# Autodesk Inventor assembly: мультипликатор
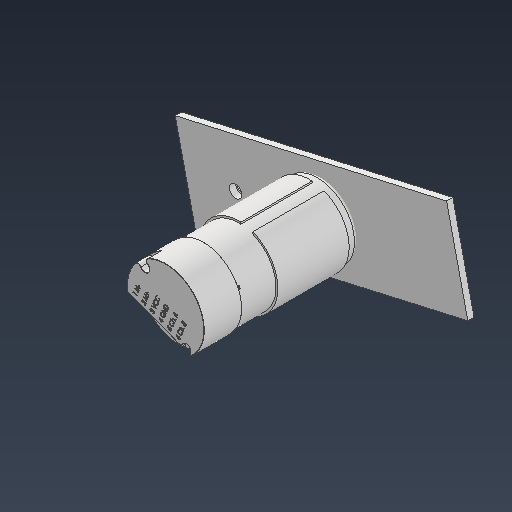
[picture p0: Inventor's stored thumbnail of the model, 512x512]
Saved by Autodesk Inventor 2025 (Build 290162000, 162)
## iProperties
Created: 2025-09-21
Part Number: мультипликатор
Document SubType Name: Assembly
Designer: GameHD
Author: GameHD
## Documents named in this file (4)
- C:\Users\GameHD\Desktop\Phantom 16950\мультипликатор.iam
- C:\Users\GameHD\Desktop\Phantom 16950\мультипликатор\Мастер проектирования\Цилиндрическое зубчатое зацепление3.iam
- C:\Users\GameHD\Desktop\Phantom 16950\пластина для редуктора.ipt
- C:\Users\GameHD\Desktop\Phantom 16950\5000-0002-0117\5000-0002-0117.iam
## Components (4 placed, 3 different names)
1. Цилиндрическое зубчатое зацепление:2 [sub-assembly] — Заподлицо:1, Совмещение:3, Заподлицо:2
2. пластина для редуктора:1 — Совмещение:1, Совмещение:2, Совмещение:3, Совмещение:4
3. 5000-0002-0117:2 [sub-assembly] — Заподлицо:1, Совмещение:1, Совмещение:2
4. Цилиндрическое зубчатое зацепление:3 [sub-assembly] — Совмещение:4, Заподлицо:2
## Relationships (6: Mate 4, Flush 2)
- Заподлицо:1 [Flush]: Цилиндрическое зубчатое зацепление:2 ↔ 5000-0002-0117:2
- Совмещение:1 [Mate]: пластина для редуктора:1 ↔ 5000-0002-0117:2
- Совмещение:2 [Mate]: пластина для редуктора:1 ↔ 5000-0002-0117:2
- Совмещение:3 [Mate]: Цилиндрическое зубчатое зацепление:2 ↔ пластина для редуктора:1
- Совмещение:4 [Mate]: пластина для редуктора:1 ↔ Цилиндрическое зубчатое зацепление:3
- Заподлицо:2 [Flush]: Цилиндрическое зубчатое зацепление:2 ↔ Цилиндрическое зубчатое зацепление:3
